# Autodesk Inventor assembly: DraftAssembly
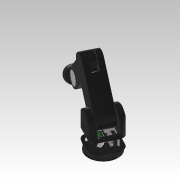
[picture p0: Inventor's stored thumbnail of the model, 180x180]
Saved by Autodesk Inventor 2020 (Build 240168000, 168)
## iProperties
Created: 2021-03-19
Part Number: DraftAssembly
Document SubType Name: Assembly
Designer: DDeGo
Author: DDeGo
## Documents named in this file (31)
- C:\Users\DDeGo\Documents\Drew\Projects\OS-ARM\cad\FirstDraft\DraftAssembly.iam
- C:\Users\DDeGo\Documents\Drew\Projects\OS-ARM\cad\FirstDraft\Base.ipt
- C:\Users\DDeGo\Documents\Drew\Projects\OS-ARM\cad\FirstDraft\Wrist.ipt
- C:\Users\DDeGo\Documents\Drew\Projects\OS-ARM\cad\FirstDraft\J1_Base.ipt
- C:\Users\DDeGo\Documents\Drew\Projects\OS-ARM\cad\OTS\Electronics\NEMA 23 - 41mm.ipt
- C:\Users\DDeGo\Documents\Drew\Projects\OS-ARM\cad\OTS\Radial Bearings\6815 bearing.ipt
- C:\Users\DDeGo\Documents\Drew\Projects\OS-ARM\cad\FirstDraft\J0_BaseMotorMount.ipt
- C:\Users\DDeGo\Documents\Drew\Projects\OS-ARM\cad\OTS\Radial Bearings\608 bearing.ipt
- C:\Users\DDeGo\Documents\Drew\Projects\OS-ARM\cad\OTS\Thrust Bearings\AXK7095 thrust bearing.ipt
- C:\Users\DDeGo\Documents\Drew\Projects\OS-ARM\cad\FirstDraft\J0_BaseMotorMount2.ipt
- C:\Users\DDeGo\Documents\Drew\Projects\OS-ARM\cad\FirstDraft\J0_DriveDisc.ipt
- C:\Users\DDeGo\Documents\Drew\Projects\OS-ARM\cad\FirstDraft\J1_NewBase.ipt
- C:\Users\DDeGo\Documents\Drew\Projects\OS-ARM\cad\OTS\Radial Bearings\6810 bearing.ipt
- C:\Users\DDeGo\Documents\Drew\Projects\OS-ARM\cad\FirstDraft\J1_NewBaseHDSide.ipt
- C:\Users\DDeGo\Documents\Drew\Projects\OS-ARM\cad\FirstDraft\SmallEncoder.ipt
- C:\Users\DDeGo\Documents\Drew\Projects\OS-ARM\cad\FirstDraft\J0_EncoderBracket.ipt
- C:\Users\DDeGo\Documents\Drew\Projects\OS-ARM\cad\FirstDraft\J0_Post.ipt
- C:\Users\DDeGo\Documents\Drew\Projects\OS-ARM\cad\OTS\Other\DiametricMagnet 1-4 x 1-8.ipt
- C:\Users\DDeGo\Documents\Drew\Projects\OS-ARM\cad\FirstDraft\DraftAssembly\Design Accelerator\Spur Gears1.iam
- C:\Users\DDeGo\Documents\Drew\Projects\OS-ARM\cad\FirstDraft\J0_DriveGear.ipt
- C:\Users\DDeGo\Documents\Drew\Projects\OS-ARM\cad\FirstDraft\DraftAssembly\Design Accelerator\Spur Gears2.iam
- C:\Users\DDeGo\Documents\Drew\Projects\OS-ARM\cad\OTS\Other\M8x160mm Threaded Rod.ipt
- C:\Users\DDeGo\Documents\Drew\Projects\OS-ARM\cad\OTS\Other\GT2 20T Drive Pulley.ipt
- C:\Users\DDeGo\Documents\Drew\Projects\OS-ARM\cad\FirstDraft\Link1.iam
- C:\Users\DDeGo\Documents\Drew\Projects\OS-ARM\cad\HarmonicDrive75mm V2\HarmonicDrive75mmV2.iam
- C:\Users\DDeGo\Documents\Drew\Projects\OS-ARM\cad\FirstDraft\J3DriveGear.ipt
- C:\Users\DDeGo\Documents\Drew\Projects\OS-ARM\cad\OTS\Other\GT2 60T Drive Pulley.ipt
- C:\Users\DDeGo\Documents\Drew\Projects\OS-ARM\cad\OTS\Radial Bearings\688 bearing.ipt
- C:\Users\DDeGo\Documents\Drew\Projects\OS-ARM\cad\FirstDraft\MotherbaordV2\OSR_Prime_V2.iam
- C:\Users\DDeGo\Documents\Drew\Projects\OS-ARM\cad\FirstDraft\Link2.iam
- C:\Users\DDeGo\Documents\Drew\Projects\OS-ARM\cad\FirstDraft\Link3.iam
## Components (33 placed, 30 different names)
1. Base:1 — Mate:57, Mate:87, Flush:11, Flush:12, Flush:13, Mate:106, Mate:107, Mate:123, Angle:4
2. Wrist:1 — Angle:4
3. J1_Base:1 — Mate:82, Mate:92, Mate:96, Mate:97, Mate:98, Mate:99, Mate:113, Mate:174, Mate:175, Mate:176, Mate:240, Mate:241, Mate:242
4. NEMA 23 - 41mm:2 — Mate:174, Mate:175, Mate:176, Mate:180
5. NEMA 23 - 41mm:3 — Mate:77, Mate:78, Mate:79, Mate:138
6. J0_BaseMotorMount:1 — Mate:57, Mate:66, Mate:67, Mate:73, Mate:74, Mate:98, Mate:99, Mate:173, Mate:185
7. 608 bearing:1 — Mate:104, Mate:132, Mate:133
8. AXK7095 thrust bearing:1 — Mate:66, Mate:67, Mate:140
9. J0_BaseMotorMount2:1 — Mate:73, Mate:74, Mate:77, Mate:78, Mate:79, Mate:82, Mate:104, Mate:124, Mate:125, Mate:126, Mate:132, Mate:185
10. J0_DriveDisc:1 — Mate:87, Mate:108, Angle:3, Mate:134, Flush:15, Mate:139, Mate:140, Rotation:1
11. J1_NewBase:1 — Mate:92, Mate:96, Mate:97, Mate:114, Mate:115, Mate:161, Mate:226, Mate:227, Mate:228, Mate:229
12. 6815 bearing:3 — Mate:178, Mate:210, Mate:211
13. 6810 bearing:1 — Mate:106, Mate:108, Mate:139
14. AXK7095 thrust bearing:2 — Mate:107, Mate:123, Mate:173
15. J1_NewBaseHDSide:1 — Mate:113, Mate:114, Mate:115, Mate:178, Mate:211, Mate:212, Mate:215
16. SmallEncoder:1 — Mate:127, Mate:128, Angle:2
17. J0_EncoderBracket:1 — Mate:124, Mate:125, Mate:126, Mate:127, Mate:128, Angle:2
18. J0_Post:1 — Mate:133, Angle:3, Mate:134, Mate:135, Mate:136
19. DiametricMagnet 1-4 x 1-8:1 — Mate:135, Mate:136
20. J0_DriveGear:1 — Mate:138, Flush:15, Rotation:1
21. J0 Drive Gears [sub-assembly]
22. J1 Encoder Gears [sub-assembly]
23. M8x160mm Threaded Rod:1 — Mate:161, Mate:186, Mate:224, Mate:225
24. GT2 20T Drive Pulley:1 — Mate:180, Flush:19
25. Link1:1 [sub-assembly] — Mate:186, Mate:213, Mate:214, Mate:244, Mate:245, Mate:246
26. HarmonicDrive75mmV2:1 [sub-assembly] — Mate:210, Mate:212, Mate:213, Mate:214, Mate:215, Mate:225
27. GT2 60T Drive Pulley:1 — Mate:224, Mate:230, Flush:19
28. 688 bearing:1 — Mate:227, Mate:229
29. 688 bearing:2 — Mate:226, Mate:228, Mate:230
30. J3DriveGear:2 — Mate:249, Mate:251
31. OSR_Prime_V2:1 [sub-assembly] — Mate:240, Mate:241, Mate:242
32. Link2:1 [sub-assembly] — Mate:244, Mate:245, Mate:246, Mate:249, Mate:251, Mate:252, Mate:253
33. Link3:1 [sub-assembly] — Mate:252, Mate:253
## Relationships (77: Mate 68, Flush 5, Angle 3, RelateRotation 1)
- Mate:57: Base:1 ↔ J0_BaseMotorMount:1
- Mate:66: J0_BaseMotorMount:1 ↔ AXK7095 thrust bearing:1
- Mate:67: J0_BaseMotorMount:1 ↔ AXK7095 thrust bearing:1
- Mate:73: J0_BaseMotorMount:1 ↔ J0_BaseMotorMount2:1
- Mate:74: J0_BaseMotorMount:1 ↔ J0_BaseMotorMount2:1
- Mate:77: NEMA 23 - 41mm:3 ↔ J0_BaseMotorMount2:1
- Mate:78: NEMA 23 - 41mm:3 ↔ J0_BaseMotorMount2:1
- Mate:79: NEMA 23 - 41mm:3 ↔ J0_BaseMotorMount2:1
- Mate:82: J1_Base:1 ↔ J0_BaseMotorMount2:1
- Mate:87: Base:1 ↔ J0_DriveDisc:1
- Mate:92: J1_Base:1 ↔ J1_NewBase:1
- Mate:96: J1_Base:1 ↔ J1_NewBase:1
- Mate:97: J1_Base:1 ↔ J1_NewBase:1
- Mate:98: J1_Base:1 ↔ J0_BaseMotorMount:1
- Mate:99: J1_Base:1 ↔ J0_BaseMotorMount:1
- Flush:11: Base:1
- Flush:12: Base:1
- Flush:13: Base:1
- Mate:104: 608 bearing:1 ↔ J0_BaseMotorMount2:1
- Mate:106: Base:1 ↔ 6810 bearing:1
- Mate:107: Base:1 ↔ AXK7095 thrust bearing:2
- Mate:108: J0_DriveDisc:1 ↔ 6810 bearing:1
- Mate:113: J1_Base:1 ↔ J1_NewBaseHDSide:1
- Mate:114: J1_NewBase:1 ↔ J1_NewBaseHDSide:1
- Mate:115: J1_NewBase:1 ↔ J1_NewBaseHDSide:1
- Mate:123: Base:1 ↔ AXK7095 thrust bearing:2
- Mate:124: J0_BaseMotorMount2:1 ↔ J0_EncoderBracket:1
- Mate:125: J0_BaseMotorMount2:1 ↔ J0_EncoderBracket:1
- Mate:126: J0_BaseMotorMount2:1 ↔ J0_EncoderBracket:1
- Mate:127: SmallEncoder:1 ↔ J0_EncoderBracket:1
- Mate:128: SmallEncoder:1 ↔ J0_EncoderBracket:1
- Angle:2 (0 deg): SmallEncoder:1 ↔ J0_EncoderBracket:1
- Mate:132: 608 bearing:1 ↔ J0_BaseMotorMount2:1
- Mate:133: 608 bearing:1 ↔ J0_Post:1
- Angle:3 (0 deg): J0_DriveDisc:1 ↔ J0_Post:1
- Mate:134: J0_DriveDisc:1 ↔ J0_Post:1
- Mate:135: J0_Post:1 ↔ DiametricMagnet 1-4 x 1-8:1
- Mate:136: J0_Post:1 ↔ DiametricMagnet 1-4 x 1-8:1
- Mate:138: NEMA 23 - 41mm:3 ↔ J0_DriveGear:1
- Flush:15: J0_DriveDisc:1 ↔ J0_DriveGear:1
- Mate:139: J0_DriveDisc:1 ↔ 6810 bearing:1
- Mate:140: AXK7095 thrust bearing:1 ↔ J0_DriveDisc:1
- Rotation:1 [RelateRotation] (0.13 ul): J0_DriveDisc:1 ↔ J0_DriveGear:1
- Mate:161 (1.5 mm): J1_NewBase:1 ↔ M8x160mm Threaded Rod:1
- Mate:173: J0_BaseMotorMount:1 ↔ AXK7095 thrust bearing:2
- Mate:174: J1_Base:1 ↔ NEMA 23 - 41mm:2
- Mate:175: J1_Base:1 ↔ NEMA 23 - 41mm:2
- Mate:176 (0.2 mm): J1_Base:1 ↔ NEMA 23 - 41mm:2
- Mate:178: 6815 bearing:3 ↔ J1_NewBaseHDSide:1
- Mate:180: NEMA 23 - 41mm:2 ↔ GT2 20T Drive Pulley:1
- Mate:185: J0_BaseMotorMount:1 ↔ J0_BaseMotorMount2:1
- Mate:186: M8x160mm Threaded Rod:1 ↔ Link1:1
- Mate:210: 6815 bearing:3 ↔ HarmonicDrive75mmV2:1
- Mate:211: 6815 bearing:3 ↔ J1_NewBaseHDSide:1
- Mate:212: J1_NewBaseHDSide:1 ↔ HarmonicDrive75mmV2:1
- Mate:213: Link1:1 ↔ HarmonicDrive75mmV2:1
- Mate:214: Link1:1 ↔ HarmonicDrive75mmV2:1
- Mate:215: J1_NewBaseHDSide:1 ↔ HarmonicDrive75mmV2:1
- Mate:224: M8x160mm Threaded Rod:1 ↔ GT2 60T Drive Pulley:1
- Mate:225: M8x160mm Threaded Rod:1 ↔ HarmonicDrive75mmV2:1
- Mate:226: J1_NewBase:1 ↔ 688 bearing:2
- Mate:227: J1_NewBase:1 ↔ 688 bearing:1
- Mate:228: J1_NewBase:1 ↔ 688 bearing:2
- Mate:229: J1_NewBase:1 ↔ 688 bearing:1
- Mate:230 (2 mm): GT2 60T Drive Pulley:1 ↔ 688 bearing:2
- Flush:19: GT2 20T Drive Pulley:1 ↔ GT2 60T Drive Pulley:1
- Mate:240: J1_Base:1 ↔ OSR_Prime_V2:1
- Mate:241: J1_Base:1 ↔ OSR_Prime_V2:1
- Mate:242: J1_Base:1 ↔ OSR_Prime_V2:1
- Mate:244: Link1:1 ↔ Link2:1
- Mate:245: Link1:1 ↔ Link2:1
- Mate:246: Link1:1 ↔ Link2:1
- Mate:249: J3DriveGear:2 ↔ Link2:1
- Angle:4 (90 deg): Base:1 ↔ Wrist:1
- Mate:251: J3DriveGear:2 ↔ Link2:1
- Mate:252: Link2:1 ↔ Link3:1
- Mate:253: Link2:1 ↔ Link3:1
